# Autodesk Inventor assembly: FE-00024
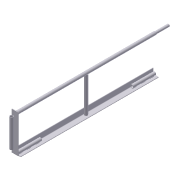
[picture p0: Inventor's stored thumbnail of the model, 180x180]
Saved by Autodesk Inventor 2012 (Build 160160000, 160)
## iProperties
Company: FIRST
Created: 2008-06-06
Part Number: FE-00024
Document SubType Name: Assembly
Designer: dfoster
Description: Field Rail Assy - Right
Title: Field Rail Assy - Right
Author: dfoster
## Documents named in this file (5)
- C:\Data Folder\FRC 2012 Field\Components\FE-00024.iam
- C:\Data Folder\FRC 2012 Field\Components\FE-00005.iam
- C:\Data Folder\FRC 2012 Field\Components\FE-00018.iam
- C:\Data Folder\FRC 2012 Field\Components\FE-00026.ipt
- C:\Data Folder\FRC 2012 Field\Components\HW-00010.ipt
## Components (9 placed, 4 different names)
1. FE-00005:1 [sub-assembly] — Mate:1, Angle:1, Mate:2, Mate:3, Tangent:1, Mate:4, Tangent:2, Angle:2, Mate:5, Flush:1, Mate:6, Tangent:3
2. FE-00018:1 [sub-assembly] — Mate:1, Angle:1, Mate:2
3. FE-00026:1 — Angle:2, Mate:5, Flush:1
4. HW-00010:2 — Mate:3, Tangent:1
5. HW-00010:4
6. HW-00010:1 — Mate:4, Tangent:2
7. HW-00010:5
8. HW-00010:3 — Mate:6, Tangent:3
9. HW-00010:6
## Component patterns: (2 elements, first: HW-00010:2), (2 elements, first: HW-00010:1), (2 elements, first: HW-00010:3)
## Relationships (12: Mate 6, Tangent 3, Angle 2, Flush 1)
- Mate:1: FE-00005:1 ↔ FE-00018:1
- Angle:1 (180 deg): FE-00005:1 ↔ FE-00018:1
- Mate:2 (6.35 mm): FE-00005:1 ↔ FE-00018:1
- Mate:3: FE-00005:1 ↔ HW-00010:2
- Tangent:1: FE-00005:1 ↔ HW-00010:2
- Mate:4: FE-00005:1 ↔ HW-00010:1
- Tangent:2: FE-00005:1 ↔ HW-00010:1
- Angle:2 (0 deg): FE-00005:1 ↔ FE-00026:1
- Mate:5: FE-00005:1 ↔ FE-00026:1
- Flush:1 (-177.8 mm): FE-00005:1 ↔ FE-00026:1
- Mate:6: FE-00005:1 ↔ HW-00010:3
- Tangent:3: FE-00005:1 ↔ HW-00010:3
